# Autodesk Inventor assembly: Carousel
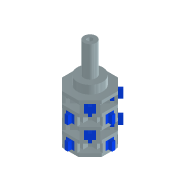
[picture p0: Inventor's stored thumbnail of the model, 180x180]
Saved by Autodesk Inventor 2021 (Build 250183000, 183)
## iProperties
Created: 2023-03-07
Part Number: Carousel
Document SubType Name: Assembly
Designer: nvladi
Author: nvladi
## Documents named in this file (4)
- C:\Users\Public\GitHub-public\benchtop-hardware\Benchtop\custom-parts\sample_handling\assemblies\Carousel.iam
- C:\Users\Public\GitHub-public\benchtop-hardware\Benchtop\custom-parts\sample_handling\carousel\MSL_base.ipt
- C:\Users\Public\GitHub-public\benchtop-hardware\Benchtop\custom-parts\sample_handling\carousel\MSL_Top.ipt
- C:\Users\Public\GitHub-public\benchtop-hardware\Benchtop\custom-parts\sample_handling\carousel\Agarose-block.ipt
## Components (15 placed, 3 different names)
1. MSL_base:1 — Insert:1, Insert:2, Angle:1, Mate:6, Flush:6, Mate:10, Flush:10
2. MSL_base:2 — Insert:3, Insert:4, Angle:2, Flush:5, Mate:5, Mate:9, Flush:9
3. MSL_base:3 — Insert:2, Insert:3, Angle:2, Mate:2, Flush:2, Mate:4, Flush:4, Mate:7, Flush:7
4. MSL_base:4 — Insert:1, Angle:1, Mate:1, Flush:1, Mate:3, Flush:3, Mate:8, Flush:8
5. MSL_Top:1 — Insert:4
6. Agarose-block:1 — Mate:1, Flush:1
7. Agarose-block:2 — Mate:2, Flush:2
8. Agarose-block:3 — Mate:6, Flush:6
9. Agarose-block:4 — Mate:4, Flush:4
10. Agarose-block:5 — Flush:5, Mate:5
11. Agarose-block:6 — Mate:3, Flush:3
12. Agarose-block:7 — Mate:7, Flush:7
13. Agarose-block:8 — Mate:8, Flush:8
14. Agarose-block:9 — Mate:9, Flush:9
15. Agarose-block:10 — Mate:10, Flush:10
## Relationships (26: Mate 10, Flush 10, Insert 4, Angle 2)
- Insert:1: MSL_base:1 ↔ MSL_base:4
- Insert:2: MSL_base:1 ↔ MSL_base:3
- Insert:3: MSL_base:2 ↔ MSL_base:3
- Insert:4 (2 mm): MSL_base:2 ↔ MSL_Top:1
- Angle:1 (45 deg): MSL_base:1 ↔ MSL_base:4
- Angle:2 (45 deg): MSL_base:2 ↔ MSL_base:3
- Mate:1: MSL_base:4 ↔ Agarose-block:1
- Flush:1: MSL_base:4 ↔ Agarose-block:1
- Mate:2: MSL_base:3 ↔ Agarose-block:2
- Flush:2: MSL_base:3 ↔ Agarose-block:2
- Mate:3: MSL_base:4 ↔ Agarose-block:6
- Flush:3: MSL_base:4 ↔ Agarose-block:6
- Mate:4: MSL_base:3 ↔ Agarose-block:4
- Flush:4: MSL_base:3 ↔ Agarose-block:4
- Flush:5: MSL_base:2 ↔ Agarose-block:5
- Mate:5: MSL_base:2 ↔ Agarose-block:5
- Mate:6: MSL_base:1 ↔ Agarose-block:3
- Flush:6: MSL_base:1 ↔ Agarose-block:3
- Mate:7: MSL_base:3 ↔ Agarose-block:7
- Flush:7: MSL_base:3 ↔ Agarose-block:7
- Mate:8: MSL_base:4 ↔ Agarose-block:8
- Flush:8: MSL_base:4 ↔ Agarose-block:8
- Mate:9: MSL_base:2 ↔ Agarose-block:9
- Flush:9: MSL_base:2 ↔ Agarose-block:9
- Mate:10: MSL_base:1 ↔ Agarose-block:10
- Flush:10: MSL_base:1 ↔ Agarose-block:10
